# Autodesk Inventor assembly: Assembled Valve Actuator
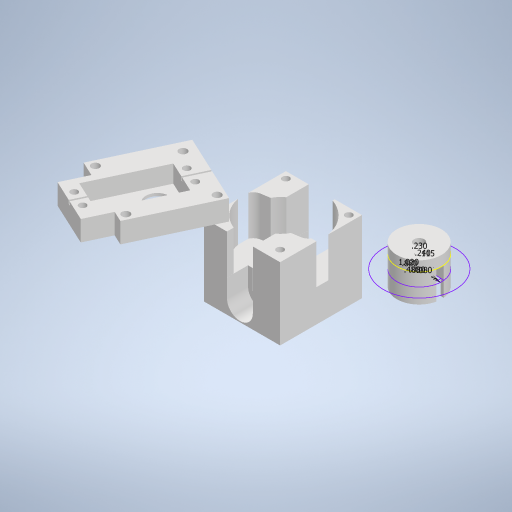
[picture p0: Inventor's stored thumbnail of the model, 512x512]
Saved by Autodesk Inventor 2024 (Build 280153000, 153)
## iProperties
Created: 2023-03-15
Part Number: Assembled Valve Actuator
Document SubType Name: Assembly
Designer: tommy
Author: tommy
## Documents named in this file (4)
- C:\Users\Tommy Rohmann\OneDrive\Projects\Microgravity-Press-Washing-Machine\Sub-System Design and Documentation\Piping Systems\Actuated Ball Valves\Assembled Valve Actuator.iam
- C:\Users\Tommy Rohmann\OneDrive\Projects\Microgravity-Press-Washing-Machine\Sub-System Design and Documentation\Piping Systems\Actuated Ball Valves\Ball Valve Mount.ipt
- C:\Users\Tommy Rohmann\OneDrive\Projects\Microgravity-Press-Washing-Machine\Sub-System Design and Documentation\Piping Systems\Actuated Ball Valves\Handle Servo Interface.ipt
- C:\Users\Tommy Rohmann\OneDrive\Projects\Microgravity-Press-Washing-Machine\Sub-System Design and Documentation\Piping Systems\Actuated Ball Valves\Servo Mount.ipt
## Components (3 placed, 3 different names)
1. Ball Valve Mount:1 — Mate:1, Mate:3, Mate:4
2. Handle Servo Interface:1 — Mate:1
3. Servo Mount:1 — Mate:3, Mate:4
## Relationships (3: Mate 3)
- Mate:1: Ball Valve Mount:1 ↔ Handle Servo Interface:1
- Mate:3: Ball Valve Mount:1 ↔ Servo Mount:1
- Mate:4: Ball Valve Mount:1 ↔ Servo Mount:1
